# Autodesk Inventor assembly: gantry
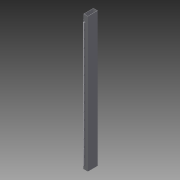
[picture p0: Inventor's stored thumbnail of the model, 180x180]
Saved by Autodesk Inventor 2013 (Build 170138000, 138)
## iProperties
Created: 2012-11-30
Part Number: gantry
Document SubType Name: Assembly
Designer: istvan.burbank
Mass: 1547.99 g
Surface Area: 9493.27 cm^2
Volume: 1547.99 cm^3
Density: 1 g/cm^3
Author: istvan.burbank
## Documents named in this file (6)
- E:\GitHub\Crown-Fire\CAD\Gantry\gantry.iam
- E:\GitHub\Crown-Fire\CAD\Gantry\gantryFrame.ipt
- E:\GitHub\Crown-Fire\CAD\Gantry\rack-x.ipt
- D:\GitHub\Crown-Fire\CAD\Templates\squareTube1.75x4.ipt
- E:\GitHub\Crown-Fire\CAD\Gantry\x-vee-track.ipt
- E:\GitHub\Crown-Fire\CAD\Templates\vee-track.ipt
## Components (4 placed, 3 different names)
1. gantryFrame:1 — Mate:1, Angle:1, Flush:2, Flush:6, Mate:2, Mate:3, Mate:4, Mate:5, Flush:7, Flush:8
2. rack-x:1 — Mate:1, Angle:1, Flush:2, Flush:6
3. x-vee-track:1 — Mate:3, Mate:4, Flush:8
4. x-vee-track:2 — Mate:2, Mate:5, Flush:7
## Relationships (10: Mate 5, Flush 4, Angle 1)
- Mate:1: gantryFrame:1 ↔ rack-x:1
- Angle:1 (0 deg): gantryFrame:1 ↔ rack-x:1
- Flush:2 (-38.1 mm): gantryFrame:1 ↔ rack-x:1
- Flush:6 (-6.35 mm): gantryFrame:1 ↔ rack-x:1
- Mate:2: gantryFrame:1 ↔ x-vee-track:2
- Mate:3: gantryFrame:1 ↔ x-vee-track:1
- Mate:4: gantryFrame:1 ↔ x-vee-track:1
- Mate:5: gantryFrame:1 ↔ x-vee-track:2
- Flush:7 (-50.8 mm): gantryFrame:1 ↔ x-vee-track:2
- Flush:8 (-50.8 mm): gantryFrame:1 ↔ x-vee-track:1
